# Autodesk Inventor assembly: ServoWithPlateCoupler
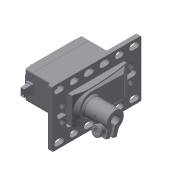
[picture p0: Inventor's stored thumbnail of the model, 180x180]
Saved by Autodesk Inventor 2018 (Build 220112000, 112)
## iProperties
Created: 2018-10-29
Part Number: ServoWithPlateCoupler
Document SubType Name: Assembly
Designer: ball
Author: ball
## Documents named in this file (3)
- C:\FTC\FTC8863CAD\2018Robot\ServoWithPlateCoupler.iam
- C:\FTC\FTC8863CAD\2018Robot\ServoWithServoPlate.iam
- C:\FTC\FTC8863CAD\GoBilda\4001 Parts\4001-0025-0006 assembly.ipt
## Components (2 placed, 2 different names)
1. ServoWithServoPlate:1 [sub-assembly] — Mate:1, Mate:2
2. 4001-0025-0006 assembly:1 — Mate:1, Mate:2
## Relationships (2: Mate 2)
- Mate:1: ServoWithServoPlate:1 ↔ 4001-0025-0006 assembly:1
- Mate:2: ServoWithServoPlate:1 ↔ 4001-0025-0006 assembly:1
